# Autodesk Inventor assembly: Battery holder w battery
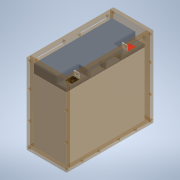
[picture p0: Inventor's stored thumbnail of the model, 180x180]
Saved by Autodesk Inventor 2022 (Build 260153000, 153)
## iProperties
Created: 2023-01-19
Part Number: Battery holder w battery
Document SubType Name: Assembly
Designer: s135320
Author: s135320
## Documents named in this file (5)
- D:\Battery holder w battery.iam
- D:\Small_Side_Piece_Final.ipt
- D:\Long_Piece_Final.ipt
- D:\Floor_Final.ipt
- D:\STEP Files\Electrical\Battery\ELEC_Battery_NP18-12B.iam
## Components (6 placed, 4 different names)
1. Small_Side_Piece:1 — Mate:5, Mate:6, Mate:12
2. Small_Side_Piece:2 — Mate:2, Mate:3, Mate:4, Mate:8
3. Long_Piece_2:1 — Mate:7, Mate:8, Mate:10
4. Long_Piece_2:2 — Mate:1, Mate:4, Mate:9
5. Floor:1 — Mate:1, Mate:2, Mate:3, Mate:5, Mate:6, Mate:7, Mate:10, Mate:11
6. ELEC_Battery_NP18-12B:1 [sub-assembly] — Mate:9, Mate:11, Mate:12
## Relationships (12: Mate 12)
- Mate:1: Long_Piece_2:2 ↔ Floor:1
- Mate:2: Small_Side_Piece:2 ↔ Floor:1
- Mate:3: Small_Side_Piece:2 ↔ Floor:1
- Mate:4: Small_Side_Piece:2 ↔ Long_Piece_2:2
- Mate:5: Small_Side_Piece:1 ↔ Floor:1
- Mate:6: Small_Side_Piece:1 ↔ Floor:1
- Mate:7: Long_Piece_2:1 ↔ Floor:1
- Mate:8: Small_Side_Piece:2 ↔ Long_Piece_2:1
- Mate:9: Long_Piece_2:2 ↔ ELEC_Battery_NP18-12B:1
- Mate:10: Long_Piece_2:1 ↔ Floor:1
- Mate:11: Floor:1 ↔ ELEC_Battery_NP18-12B:1
- Mate:12: Small_Side_Piece:1 ↔ ELEC_Battery_NP18-12B:1
